# Autodesk Inventor assembly: ArmAssembly
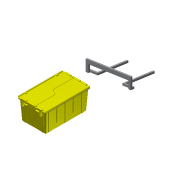
[picture p0: Inventor's stored thumbnail of the model, 180x180]
Saved by Autodesk Inventor 2015 (Build 190159000, 159)
## iProperties
Created: 2015-03-07
Part Number: ArmAssembly
Document SubType Name: Assembly
Designer: Jaden
Author: Jaden
## Documents named in this file (6)
- E:\ReDesign\ArmAssembly.iam
- E:\ReDesign\ArmBar.ipt
- E:\ReDesign\Imported Components\YELLOW_TOTEASM_ASM\YELLOW_TOTEASM_ASM.iam
- E:\ReDesign\ArmCrossBeam.ipt
- E:\ReDesign\ArmVert.ipt
- E:\ReDesign\armHorzi.ipt
## Components (8 placed, 5 different names)
1. YELLOW_TOTEASM_ASM:1 [sub-assembly]
2. ArmCrossBeam:1 — Mate:10, Mate:11, Mate:12, Mate:13
3. ArmVert:1 — Mate:10, Mate:11, Mate:14, Mate:15
4. ArmVert:2 — Mate:12, Mate:13, Mate:16, Mate:17
5. armHorzi:1 — Mate:14, Mate:15, Mate:21, Mate:22, Mate:23
6. armHorzi:2 — Mate:16, Mate:17, Mate:18, Mate:19, Mate:20
7. ArmBar:1 — Mate:18, Mate:19, Mate:20
8. ArmBar:2 — Mate:21, Mate:22, Mate:23
## Relationships (14: Mate 14)
- Mate:10: ArmCrossBeam:1 ↔ ArmVert:1
- Mate:11: ArmCrossBeam:1 ↔ ArmVert:1
- Mate:12: ArmCrossBeam:1 ↔ ArmVert:2
- Mate:13: ArmCrossBeam:1 ↔ ArmVert:2
- Mate:14: ArmVert:1 ↔ armHorzi:1
- Mate:15: ArmVert:1 ↔ armHorzi:1
- Mate:16: ArmVert:2 ↔ armHorzi:2
- Mate:17: ArmVert:2 ↔ armHorzi:2
- Mate:18: armHorzi:2 ↔ ArmBar:1
- Mate:19: armHorzi:2 ↔ ArmBar:1
- Mate:20: armHorzi:2 ↔ ArmBar:1
- Mate:21: armHorzi:1 ↔ ArmBar:2
- Mate:22: armHorzi:1 ↔ ArmBar:2
- Mate:23: armHorzi:1 ↔ ArmBar:2
